# Autodesk Inventor assembly: project1-assembly
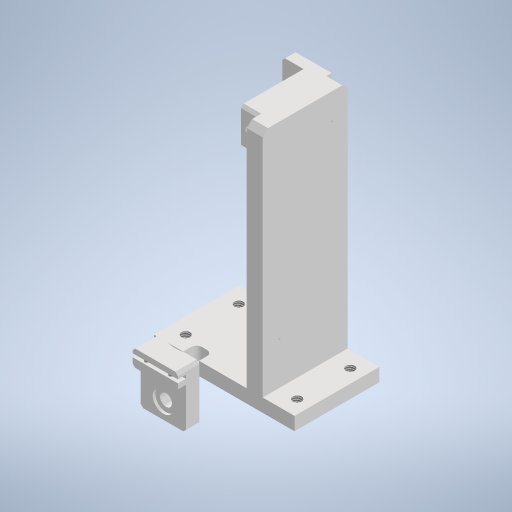
[picture p0: Inventor's stored thumbnail of the model, 512x512]
Saved by Autodesk Inventor 2024.2 (Build 282272000, 272)
## iProperties
Created: 2024-02-21
Part Number: project1-assembly
Document SubType Name: Assembly
Designer: fabig
Author: fabig
## Documents named in this file (4)
- C:\Users\fabig\OneDrive\Documents\GitHub\Git Scheme testing\Parent-folder-table-assembly-\Subproject assemblies\project1-assembly\project1-assembly.iam
- C:\Users\fabig\OneDrive\Documents\GitHub\Git Scheme testing\Parent-folder-table-assembly-\Subproject assemblies\project1-assembly\pegboard-maker-adapter\misc\ADAPTER_shutter\ADAPTER_shutter.ipt
- C:\Users\fabig\OneDrive\Documents\GitHub\Git Scheme testing\Parent-folder-table-assembly-\Subproject assemblies\project1-assembly\pegboard-maker-adapter\misc\ADAPTER_periscope\ADAPTER_periscope.ipt
- C:\Users\fabig\OneDrive\Documents\GitHub\Git Scheme testing\Parent-folder-table-assembly-\Subproject assemblies\project1-assembly\pegboard-maker-adapter\misc\ADAPTER_dichroic\ADAPTER_dichroic.ipt
## Components (3 placed, 3 different names)
1. ADAPTER_shutter:1 — Flush:1, Flush:2, Flush:3, Mate:1, Flush:4, Flush:5
2. ADAPTER_periscope:1 — Mate:1, Flush:4, Flush:5, Mate:2, Flush:6, Flush:7
3. ADAPTER_dichroic:1 — Mate:2, Flush:6, Flush:7
## Relationships (9: Flush 7, Mate 2)
- Flush:1: ADAPTER_shutter:1
- Flush:2: ADAPTER_shutter:1
- Flush:3: ADAPTER_shutter:1
- Mate:1: ADAPTER_shutter:1 ↔ ADAPTER_periscope:1
- Flush:4: ADAPTER_shutter:1 ↔ ADAPTER_periscope:1
- Flush:5: ADAPTER_shutter:1 ↔ ADAPTER_periscope:1
- Mate:2: ADAPTER_periscope:1 ↔ ADAPTER_dichroic:1
- Flush:6: ADAPTER_periscope:1 ↔ ADAPTER_dichroic:1
- Flush:7: ADAPTER_periscope:1 ↔ ADAPTER_dichroic:1
